# Autodesk Inventor assembly: B_Legs0
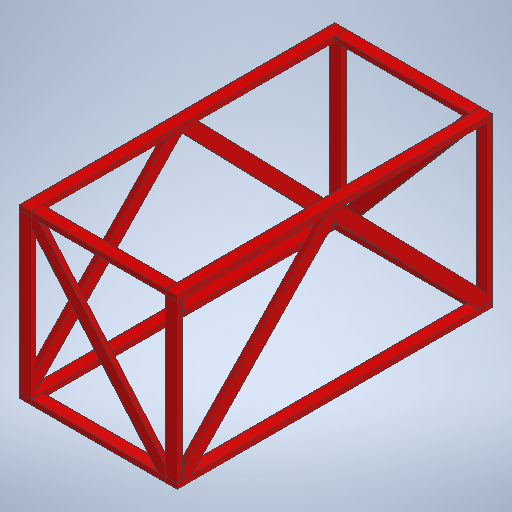
[picture p0: Inventor's stored thumbnail of the model, 512x512]
Saved by Autodesk Inventor 2025.1 (Build 291241020, 241B)
## iProperties
Created: 2024-09-19
Part Number: B_Legs0
Document SubType Name: Assembly
Designer: User
Author: User
## Documents named in this file (6)
- C:\Users\User\Documents\Tburn24\B_Legs0\B_Legs0.iam
- C:\Users\User\Documents\Tburn24\B_Legs0\8'x2x4.ipt
- C:\Users\User\Documents\Tburn24\B_Legs0\3'5x2x4.ipt
- C:\Users\User\Documents\Tburn24\B_Legs0\4x2x4.ipt
- C:\Users\User\Documents\Tburn24\B_Legs0\48x2x4-2.ipt
- C:\Users\User\Documents\Tburn24\B_Legs0\44x2x4.ipt
## Components (16 placed, 5 different names)
1. 8'x2x4:1 — Flush:1, Flush:2, Flush:3, Flush:4, Flush:5, Flush:8, Mate:3, Flush:10, Flush:12, Flush:13, Flush:14
2. 8'x2x4:2 — Mate:1, Flush:1, Flush:2, Flush:3, Mate:2, Flush:6, Flush:7, Mate:5, Flush:9, Flush:11, Flush:15, Flush:16
3. 3'5x2x4:1 — Flush:4, Flush:5
4. 3'5x2x4:2 — Mate:2, Flush:6, Flush:7, Mate:4
5. 4x2x4:1 — Flush:8, Flush:13, Flush:14, Mate:7, Flush:17, Flush:20
6. 4x2x4:2 — Mate:5, Flush:15, Flush:16, Mate:6, Flush:18, Flush:19, Flush:27
7. 4x2x4:3 — Mate:4, Flush:9, Flush:11, Mate:11
8. 4x2x4:4 — Mate:3, Flush:10, Flush:12, Mate:13, Flush:28
9. 8'x2x4:3 — Mate:7, Flush:17, Flush:20, Mate:8, Mate:9, Flush:23, Flush:24, Flush:25
10. 8'x2x4:4 — Mate:6, Flush:18, Flush:19, Flush:21, Flush:22, Flush:26, Mate:10
11. 3'5x2x4:3 — Mate:8, Flush:21, Flush:22, Mate:12
12. 3'5x2x4:4 — Mate:9, Flush:23, Flush:24
13. 48x2x4-2:1 — Flush:25
14. 48x2x4-2:2 — Flush:26, Mate:10, Mate:11
15. 44x2x4:1 — Flush:27
16. 44x2x4:2 — Mate:12, Mate:13, Flush:28
## Relationships (41: Flush 28, Mate 13)
- Mate:1: 8'x2x4:2
- Flush:1: 8'x2x4:1 ↔ 8'x2x4:2
- Flush:2 (1130.3 mm): 8'x2x4:1 ↔ 8'x2x4:2
- Flush:3: 8'x2x4:1 ↔ 8'x2x4:2
- Flush:4: 8'x2x4:1 ↔ 3'5x2x4:1
- Flush:5: 8'x2x4:1 ↔ 3'5x2x4:1
- Mate:2: 8'x2x4:2 ↔ 3'5x2x4:2
- Flush:6: 8'x2x4:2 ↔ 3'5x2x4:2
- Flush:7: 8'x2x4:2 ↔ 3'5x2x4:2
- Flush:8: 8'x2x4:1 ↔ 4x2x4:1
- Mate:3: 8'x2x4:1 ↔ 4x2x4:4
- Mate:4: 3'5x2x4:2 ↔ 4x2x4:3
- Mate:5: 8'x2x4:2 ↔ 4x2x4:2
- Flush:9: 8'x2x4:2 ↔ 4x2x4:3
- Flush:10: 8'x2x4:1 ↔ 4x2x4:4
- Flush:11: 8'x2x4:2 ↔ 4x2x4:3
- Flush:12: 8'x2x4:1 ↔ 4x2x4:4
- Flush:13: 8'x2x4:1 ↔ 4x2x4:1
- Flush:14: 8'x2x4:1 ↔ 4x2x4:1
- Flush:15: 8'x2x4:2 ↔ 4x2x4:2
- Flush:16: 8'x2x4:2 ↔ 4x2x4:2
- Mate:6: 4x2x4:2 ↔ 8'x2x4:4
- Mate:7: 4x2x4:1 ↔ 8'x2x4:3
- Flush:17: 4x2x4:1 ↔ 8'x2x4:3
- Flush:18: 4x2x4:2 ↔ 8'x2x4:4
- Flush:19: 4x2x4:2 ↔ 8'x2x4:4
- Flush:20: 4x2x4:1 ↔ 8'x2x4:3
- Mate:8: 8'x2x4:3 ↔ 3'5x2x4:3
- Mate:9: 8'x2x4:3 ↔ 3'5x2x4:4
- Flush:21: 8'x2x4:4 ↔ 3'5x2x4:3
- Flush:22: 8'x2x4:4 ↔ 3'5x2x4:3
- Flush:23: 8'x2x4:3 ↔ 3'5x2x4:4
- Flush:24: 8'x2x4:3 ↔ 3'5x2x4:4
- Flush:25: 8'x2x4:3 ↔ 48x2x4-2:1
- Flush:26: 8'x2x4:4 ↔ 48x2x4-2:2
- Mate:10: 8'x2x4:4 ↔ 48x2x4-2:2
- Mate:11: 4x2x4:3 ↔ 48x2x4-2:2
- Flush:27: 4x2x4:2 ↔ 44x2x4:1
- Mate:12: 3'5x2x4:3 ↔ 44x2x4:2
- Mate:13: 4x2x4:4 ↔ 44x2x4:2
- Flush:28: 4x2x4:4 ↔ 44x2x4:2
